# Autodesk Inventor assembly: TorsoUnit
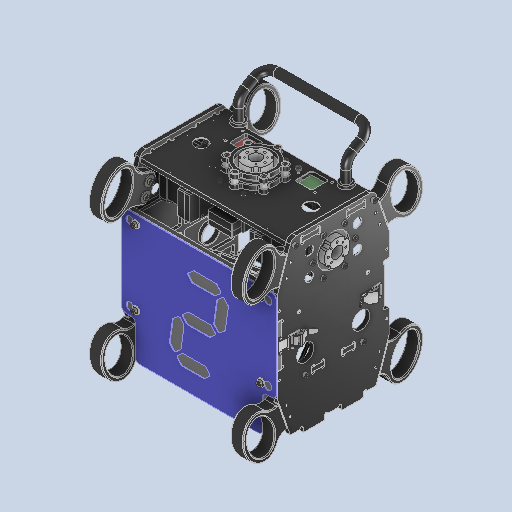
[picture p0: Inventor's stored thumbnail of the model, 512x512]
Saved by Autodesk Inventor 2024.2 (Build 282272000, 272)
## iProperties
Created: 2024-01-05
Part Number: TorsoUnit
Document SubType Name: Assembly
Designer: Masato Kubotera
Mass: 1646.85 g
Surface Area: 4802.66 cm^2
Volume: 709.254 cm^3
Author: Masato Kubotera
## Documents named in this file (24)
- C:\Users\masato\OneDrive - Chiba Institute of Technology\CIT Brains\RoboCup2024\SUSTAINA-OP2-DEV\NativeFiles\Boby\Torso\TorsoUnit.iam
- C:\Users\masato\OneDrive - Chiba Institute of Technology\CIT Brains\RoboCup2024\SUSTAINA-OP2-DEV\NativeFiles\Boby\CommonDesignedComponents\CrossRollerBearingUnit\CrossRollerBearingUnit.iam
- C:\Users\masato\OneDrive - Chiba Institute of Technology\CIT Brains\RoboCup2024\SUSTAINA-OP2-DEV\NativeFiles\Boby\COTS\Actuators\PMX-SCR-5204HV.ipt
- C:\Users\masato\OneDrive - Chiba Institute of Technology\CIT Brains\RoboCup2024\SUSTAINA-OP2-DEV\NativeFiles\Boby\Torso\TorsoUpperFrame.ipt
- C:\Users\masato\OneDrive - Chiba Institute of Technology\CIT Brains\RoboCup2024\SUSTAINA-OP2-DEV\NativeFiles\Boby\COTS\Washers\Metal\UZB.ipt
- C:\Users\masato\OneDrive - Chiba Institute of Technology\CIT Brains\RoboCup2024\SUSTAINA-OP2-DEV\NativeFiles\Boby\COTS\MisumiComponents\UHFNB125.ipt
- C:\Users\masato\OneDrive - Chiba Institute of Technology\CIT Brains\RoboCup2024\SUSTAINA-OP2-DEV\NativeFiles\Boby\COTS\Screws\CapScrew\UC-0515.ipt
- C:\Users\masato\OneDrive - Chiba Institute of Technology\CIT Brains\RoboCup2024\SUSTAINA-OP2-DEV\NativeFiles\Boby\COTS\Screws\CapScrew\FC-2615EB.ipt
- C:\Users\masato\OneDrive - Chiba Institute of Technology\CIT Brains\RoboCup2024\SUSTAINA-OP2-DEV\NativeFiles\Boby\Torso\TorsoFrontCoverFrame.ipt
- C:\Users\masato\OneDrive - Chiba Institute of Technology\CIT Brains\RoboCup2024\SUSTAINA-OP2-DEV\NativeFiles\Boby\Torso\TorsoColorMarker.ipt
- C:\Users\masato\OneDrive - Chiba Institute of Technology\CIT Brains\RoboCup2024\SUSTAINA-OP2-DEV\NativeFiles\Boby\Torso\TorsoLowerFrame.ipt
- C:\Users\masato\OneDrive - Chiba Institute of Technology\CIT Brains\RoboCup2024\SUSTAINA-OP2-DEV\NativeFiles\Boby\CustomPCBs\SUSTAINA-BUTTON-MODULE.ipt
- C:\Users\masato\OneDrive - Chiba Institute of Technology\CIT Brains\RoboCup2024\SUSTAINA-OP2-DEV\NativeFiles\Boby\COTS\Screws\CapScrew\PCC-0306.ipt
- C:\Users\masato\OneDrive - Chiba Institute of Technology\CIT Brains\RoboCup2024\SUSTAINA-OP2-DEV\NativeFiles\Boby\COTS\ElectronicComponents\DK-42688-P\DK-42688-P.ipt
- C:\Users\masato\OneDrive - Chiba Institute of Technology\CIT Brains\RoboCup2024\SUSTAINA-OP2-DEV\NativeFiles\Boby\COTS\Bushes\D2030-5805B.ipt
- C:\Users\masato\OneDrive - Chiba Institute of Technology\CIT Brains\RoboCup2024\SUSTAINA-OP2-DEV\NativeFiles\Boby\COTS\MisumiComponents\PKWS1\PKWS1_s.ipt
- C:\Users\masato\OneDrive - Chiba Institute of Technology\CIT Brains\RoboCup2024\SUSTAINA-OP2-DEV\NativeFiles\Boby\COTS\Screws\U-0205.ipt
- C:\Users\masato\OneDrive - Chiba Institute of Technology\CIT Brains\RoboCup2024\SUSTAINA-OP2-DEV\NativeFiles\Boby\Torso\RightTorsoSideUnit.iam
- C:\Users\masato\OneDrive - Chiba Institute of Technology\CIT Brains\RoboCup2024\SUSTAINA-OP2-DEV\NativeFiles\Boby\COTS\Bushes\L3040-8115TB.ipt
- C:\Users\masato\OneDrive - Chiba Institute of Technology\CIT Brains\RoboCup2024\SUSTAINA-OP2-DEV\NativeFiles\Boby\COTS\Screws\CapScrew\UC-0306.ipt
- C:\Users\masato\OneDrive - Chiba Institute of Technology\CIT Brains\RoboCup2024\SUSTAINA-OP2-DEV\NativeFiles\Boby\Torso\LeftTorsoSideUnit.iam
- C:\Users\masato\OneDrive - Chiba Institute of Technology\CIT Brains\RoboCup2024\SUSTAINA-OP2-DEV\NativeFiles\Boby\COTS\Screws\CapScrew\UC-0206.ipt
- C:\Users\masato\OneDrive - Chiba Institute of Technology\CIT Brains\RoboCup2024\SUSTAINA-OP2-DEV\NativeFiles\Boby\Torso\TorsoButtonLowerCoverFrame.ipt
- C:\Users\masato\OneDrive - Chiba Institute of Technology\CIT Brains\RoboCup2024\SUSTAINA-OP2-DEV\NativeFiles\Boby\Torso\TorsoButtonUpperCoverFrame.ipt
## Components (45 placed, 23 different names)
1. CrossRollerBearingUnit:1 [sub-assembly] — Mate:1, Flush:3, Mate:2, Insert:152, Insert:153
2. LeftTorsoSideUnit:1 [sub-assembly] — Insert:254, Insert:255, Insert:258, Insert:259, Mate:209, Flush:5, Flush:4
3. RightTorsoSideUnit:1 [sub-assembly] — Insert:256, Insert:257, Insert:260, Insert:261
4. TorsoButtonLowerCoverFrame:1 — Insert:307, Insert:308, Insert:309, Insert:310
5. TorsoButtonUpperCoverFrame:1 — Insert:303, Insert:304, Insert:305, Insert:306, Flush:211, Flush:212, Mate:210, Insert:307, Insert:308, Insert:309, Insert:310
6. UHFNB125:1 — Insert:9, Insert:10
7. DK-42688-P:1 — Mate:206, Mate:207, Mate:208
8. PKWS1_s:3 — Insert:289, Insert:290
9. PKWS1_s:4 — Insert:291, Insert:292
10. TorsoFrontCoverFrame:1 — Mate:209, Flush:4, Flush:5, Insert:289, Insert:290, Insert:291, Insert:292, Insert:294, Insert:298, Insert:299, Insert:300
11. TorsoUpperFrame:1 — Insert:152, Insert:153, Insert:154, Insert:155, Insert:156, Insert:157, Insert:158, Insert:159, Insert:160, Insert:161, Insert:218, Insert:219, Insert:220, Insert:221, Insert:254, Insert:255, Insert:256, Insert:257, Insert:303, Insert:304, Insert:305, Insert:306
12. TorsoLowerFrame:1 — Mate:206, Mate:207, Mate:208, Insert:244, Insert:245, Insert:246, Insert:247, Insert:258, Insert:259, Insert:260, Insert:261
13. SUSTAINA-BUTTON-MODULE:1 — Flush:211, Flush:212, Mate:210
14. TorsoColorMarker:1 — Insert:301, Insert:302
15. PMX-SCR-5204HV:2 — Insert:154, Insert:155
16. L3040-8115TB:4 — Insert:299
17. L3040-8115TB:1 — Insert:294, Insert:302
18. L3040-8115TB:2 — Insert:298, Insert:301
19. L3040-8115TB:3 — Insert:300
20. D2030-5805B:1 — Insert:244, Insert:248
21. D2030-5805B:4 — Insert:247, Insert:251
22. D2030-5805B:2 — Insert:245, Insert:249
23. D2030-5805B:3 — Insert:246, Insert:250
24. U-0205:5
25. U-0205:8
26. U-0205:7
27. U-0205:6
28. UC-0306:1
29. UC-0306:4
30. UC-0306:3
31. UC-0306:2
32. UC-0206:2 — Insert:248
33. UC-0206:4 — Insert:249
34. UC-0206:3 — Insert:250
35. UC-0206:1 — Insert:251
36. UC-0515:1 — Insert:161
37. UC-0515:2 — Insert:160
38. FC-2615EB:3 — Insert:156
39. FC-2615EB:4 — Insert:157
40. PCC-0306:1 — Insert:218
41. PCC-0306:2 — Insert:219
42. PCC-0306:3 — Insert:220
43. PCC-0306:4 — Insert:221
44. UZB:1 — Insert:9, Insert:158
45. UZB:2 — Insert:10, Insert:159
## Relationships (70: Insert 58, Mate 7, Flush 5)
- Insert:9: UHFNB125:1 ↔ UZB:1
- Insert:10: UHFNB125:1 ↔ UZB:2
- Mate:1: CrossRollerBearingUnit:1
- Flush:3: CrossRollerBearingUnit:1
- Mate:2: CrossRollerBearingUnit:1
- Insert:152: CrossRollerBearingUnit:1 ↔ TorsoUpperFrame:1
- Insert:153: CrossRollerBearingUnit:1 ↔ TorsoUpperFrame:1
- Insert:154: TorsoUpperFrame:1 ↔ PMX-SCR-5204HV:2
- Insert:155: TorsoUpperFrame:1 ↔ PMX-SCR-5204HV:2
- Insert:156: TorsoUpperFrame:1 ↔ FC-2615EB:3
- Insert:157: TorsoUpperFrame:1 ↔ FC-2615EB:4
- Insert:158: TorsoUpperFrame:1 ↔ UZB:1
- Insert:159: TorsoUpperFrame:1 ↔ UZB:2
- Insert:160: TorsoUpperFrame:1 ↔ UC-0515:2
- Insert:161: TorsoUpperFrame:1 ↔ UC-0515:1
- Insert:218 (3 mm): TorsoUpperFrame:1 ↔ PCC-0306:1
- Insert:219 (3 mm): TorsoUpperFrame:1 ↔ PCC-0306:2
- Insert:220 (3 mm): TorsoUpperFrame:1 ↔ PCC-0306:3
- Insert:221 (3 mm): TorsoUpperFrame:1 ↔ PCC-0306:4
- Mate:206: DK-42688-P:1 ↔ TorsoLowerFrame:1
- Mate:207: DK-42688-P:1 ↔ TorsoLowerFrame:1
- Mate:208: DK-42688-P:1 ↔ TorsoLowerFrame:1
- Insert:244: TorsoLowerFrame:1 ↔ D2030-5805B:1
- Insert:245: TorsoLowerFrame:1 ↔ D2030-5805B:2
- Insert:246: TorsoLowerFrame:1 ↔ D2030-5805B:3
- Insert:247: TorsoLowerFrame:1 ↔ D2030-5805B:4
- Insert:248: D2030-5805B:1 ↔ UC-0206:2
- Insert:249: D2030-5805B:2 ↔ UC-0206:4
- Insert:250: D2030-5805B:3 ↔ UC-0206:3
- Insert:251: D2030-5805B:4 ↔ UC-0206:1
- Insert:254: LeftTorsoSideUnit:1 ↔ TorsoUpperFrame:1
- Insert:255: LeftTorsoSideUnit:1 ↔ TorsoUpperFrame:1
- Insert:256: RightTorsoSideUnit:1 ↔ TorsoUpperFrame:1
- Insert:257: RightTorsoSideUnit:1 ↔ TorsoUpperFrame:1
- Insert:258: LeftTorsoSideUnit:1 ↔ TorsoLowerFrame:1
- Insert:259: LeftTorsoSideUnit:1 ↔ TorsoLowerFrame:1
- Insert:260: RightTorsoSideUnit:1 ↔ TorsoLowerFrame:1
- Insert:261: RightTorsoSideUnit:1 ↔ TorsoLowerFrame:1
- [Insert]: PKWS1_s:3 ↔ U-0205:5
- [Insert]: PKWS1_s:3 ↔ U-0205:6
- [Insert]: PKWS1_s:4 ↔ U-0205:7
- [Insert]: PKWS1_s:4 ↔ U-0205:8
- Mate:209: LeftTorsoSideUnit:1 ↔ TorsoFrontCoverFrame:1
- Flush:4: LeftTorsoSideUnit:1 ↔ TorsoFrontCoverFrame:1
- Flush:5: LeftTorsoSideUnit:1 ↔ TorsoFrontCoverFrame:1
- Insert:289: PKWS1_s:3 ↔ TorsoFrontCoverFrame:1
- Insert:290: PKWS1_s:3 ↔ TorsoFrontCoverFrame:1
- Insert:291: PKWS1_s:4 ↔ TorsoFrontCoverFrame:1
- Insert:292: PKWS1_s:4 ↔ TorsoFrontCoverFrame:1
- [Insert]: L3040-8115TB:1 ↔ UC-0306:1
- Insert:294: TorsoFrontCoverFrame:1 ↔ L3040-8115TB:1
- [Insert]: L3040-8115TB:2 ↔ UC-0306:2
- [Insert]: L3040-8115TB:3 ↔ UC-0306:3
- [Insert]: L3040-8115TB:4 ↔ UC-0306:4
- Insert:298: TorsoFrontCoverFrame:1 ↔ L3040-8115TB:2
- Insert:299: TorsoFrontCoverFrame:1 ↔ L3040-8115TB:4
- Insert:300: TorsoFrontCoverFrame:1 ↔ L3040-8115TB:3
- Insert:301: TorsoColorMarker:1 ↔ L3040-8115TB:2
- Insert:302: TorsoColorMarker:1 ↔ L3040-8115TB:1
- Insert:303: TorsoButtonUpperCoverFrame:1 ↔ TorsoUpperFrame:1
- Insert:304: TorsoButtonUpperCoverFrame:1 ↔ TorsoUpperFrame:1
- Insert:305: TorsoButtonUpperCoverFrame:1 ↔ TorsoUpperFrame:1
- Insert:306: TorsoButtonUpperCoverFrame:1 ↔ TorsoUpperFrame:1
- Flush:211: TorsoButtonUpperCoverFrame:1 ↔ SUSTAINA-BUTTON-MODULE:1
- Flush:212: TorsoButtonUpperCoverFrame:1 ↔ SUSTAINA-BUTTON-MODULE:1
- Mate:210: TorsoButtonUpperCoverFrame:1 ↔ SUSTAINA-BUTTON-MODULE:1
- Insert:307: TorsoButtonLowerCoverFrame:1 ↔ TorsoButtonUpperCoverFrame:1
- Insert:308: TorsoButtonLowerCoverFrame:1 ↔ TorsoButtonUpperCoverFrame:1
- Insert:309: TorsoButtonLowerCoverFrame:1 ↔ TorsoButtonUpperCoverFrame:1
- Insert:310: TorsoButtonLowerCoverFrame:1 ↔ TorsoButtonUpperCoverFrame:1
## Named parameters: d341_d132 = 0 mm, d342_d133 = 0 mm, d343_d332_d132 = 0 mm, d344_d333_d133 = 0 mm, d67_d34 = 0 mm, d373_d67_d34 = 0 mm, d374_d67_d34 = 0 mm, d375_d67_d34 = 0 mm
